# Autodesk Inventor assembly: Base Hinge and bracket
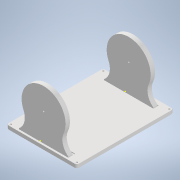
[picture p0: Inventor's stored thumbnail of the model, 180x180]
Saved by Autodesk Inventor 2020.2 (Build 242310000, 310)
## iProperties
Created: 2020-03-30
Part Number: Base Hinge and bracket
Document SubType Name: Assembly
Designer: Amaan Khalid
Author: Amaan Khalid
## Documents named in this file (3)
- C:\Users\Amaan Khalid\Desktop\Robotic Arm project\My parts\Base Hinge and bracket.iam
- C:\Users\Amaan Khalid\Desktop\Robotic Arm project\My parts\Base Bracket 1x.ipt
- C:\Users\Amaan Khalid\Desktop\Robotic Arm project\My parts\Base Hinge 2x.ipt
## Components (3 placed, 2 different names)
1. Base Bracket 1x:1 — Mate:1, Mate:2
2. Base Hinge 2x:1 — Mate:1
3. Base Hinge 2x:2 — Mate:2
## Relationships (2: Mate 2)
- Mate:1: Base Bracket 1x:1 ↔ Base Hinge 2x:1
- Mate:2: Base Bracket 1x:1 ↔ Base Hinge 2x:2
